# Autodesk Inventor assembly: toggle switch
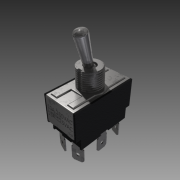
[picture p0: Inventor's stored thumbnail of the model, 180x180]
Saved by Autodesk Inventor 2012 (Build 160160000, 160)
## iProperties
Created: 2014-01-27
Part Number: toggle switch
Document SubType Name: Assembly
Designer: Michał
Author: Michał
## Documents named in this file (5)
- G:\Moje Dokumenty\Inventor\toggle switch\toggle switch.iam
- G:\Moje Dokumenty\Inventor\toggle switch\01.ipt
- G:\Moje Dokumenty\Inventor\toggle switch\02.ipt
- G:\Moje Dokumenty\Inventor\toggle switch\03.ipt
- G:\Moje Dokumenty\Inventor\toggle switch\04.ipt
## Components (9 placed, 4 different names)
1. 01:1 — Mate:1
2. 02:1 — Mate:1, Mate:2, Mate:3, Mate:4
3. 03:1 — Mate:2, Mate:3, Mate:4, Mate:5, Insert:1, Insert:2, Insert:3, Insert:4, Insert:5, Insert:6, Mate:6, Mate:7, Mate:8, Mate:9, Mate:10
4. 04:1 — Mate:5, Insert:1
5. 04:2 — Insert:2, Mate:9
6. 04:3 — Insert:3, Mate:10
7. 04:4 — Insert:4, Mate:6
8. 04:5 — Insert:5, Mate:7
9. 04:6 — Insert:6, Mate:8
## Relationships (16: Mate 10, Insert 6)
- Mate:1: 01:1 ↔ 02:1
- Mate:2: 02:1 ↔ 03:1
- Mate:3: 02:1 ↔ 03:1
- Mate:4 (0.25 mm): 02:1 ↔ 03:1
- Mate:5: 03:1 ↔ 04:1
- Insert:1: 03:1 ↔ 04:1
- Insert:2: 03:1 ↔ 04:2
- Insert:3: 03:1 ↔ 04:3
- Insert:4: 03:1 ↔ 04:4
- Insert:5: 03:1 ↔ 04:5
- Insert:6: 03:1 ↔ 04:6
- Mate:6: 03:1 ↔ 04:4
- Mate:7: 03:1 ↔ 04:5
- Mate:8: 03:1 ↔ 04:6
- Mate:9: 03:1 ↔ 04:2
- Mate:10: 03:1 ↔ 04:3
